# Autodesk Inventor assembly: 14inLift
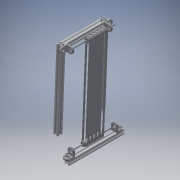
[picture p0: Inventor's stored thumbnail of the model, 180x180]
Saved by Autodesk Inventor 2016 (Build 200138000, 138)
## iProperties
Created: 2016-12-21
Part Number: 14inLift
Document SubType Name: Assembly
Designer: RoboticsUser
Author: RoboticsUser
## Documents named in this file (6)
- C:\Robotics\CAD\2016-17_CAD\14inLift - Copy.iam
- C:\Robotics\CAD\COTSParts\Bosch Extrusion\Bosch 20x20 16.66 -.ipt
- C:\Robotics\CAD\COTSParts\Actobotics\545 parts\545400_MIR.ipt
- C:\Robotics\CAD\COTSParts\Bosch Extrusion\Bosch 20x20 9 in actual.ipt
- C:\Robotics\CAD\2016-17_CAD\12inlift.iam
- C:\Robotics\CAD\COTSParts\Bosch Extrusion\Bosch 20x20 9 real.ipt
## Components (9 placed, 5 different names)
1. Bosch 20x20 16.66 -:1 — Mate:9, Mate:13, Flush:12, Flush:13, Flush:23, Flush:24, Flush:25
2. Bosch 20x20 16.66 -:2 — Mate:12, Mate:14, Flush:16, Flush:17, Flush:20, Flush:21, Flush:22
3. 545400_MIR:1 — Mate:21, Mate:22, Mate:23, Flush:27
4. 545400_MIR:2 — Mate:9, Flush:18, Flush:23
5. 545400_MIR:3 — Mate:19, Flush:19, Mate:20, Flush:26, Flush:28
6. 545400_MIR:4 — Mate:12, Flush:17, Flush:21, Flush:29, Mate:24
7. Bosch 20x20 9 in actual:1 — Mate:13, Flush:12, Flush:13, Mate:14, Flush:16, Flush:18, Flush:20, Flush:22, Flush:24, Flush:25
8. 12inlift:1 [sub-assembly] — Mate:22, Mate:23, Flush:28, Flush:29, Mate:24
9. Bosch 20x20 9 real:1 — Mate:19, Flush:19, Mate:20, Mate:21, Flush:26, Flush:27
## Relationships (26: Flush 16, Mate 10)
- Mate:9: Bosch 20x20 16.66 -:1 ↔ 545400_MIR:2
- Mate:12: Bosch 20x20 16.66 -:2 ↔ 545400_MIR:4
- Mate:13: Bosch 20x20 16.66 -:1 ↔ Bosch 20x20 9 in actual:1
- Flush:12: Bosch 20x20 16.66 -:1 ↔ Bosch 20x20 9 in actual:1
- Flush:13: Bosch 20x20 16.66 -:1 ↔ Bosch 20x20 9 in actual:1
- Mate:14: Bosch 20x20 16.66 -:2 ↔ Bosch 20x20 9 in actual:1
- Flush:16: Bosch 20x20 16.66 -:2 ↔ Bosch 20x20 9 in actual:1
- Flush:17: Bosch 20x20 16.66 -:2 ↔ 545400_MIR:4
- Flush:18: 545400_MIR:2 ↔ Bosch 20x20 9 in actual:1
- Mate:19: 545400_MIR:3 ↔ Bosch 20x20 9 real:1
- Flush:19: 545400_MIR:3 ↔ Bosch 20x20 9 real:1
- Mate:20 (-12.7 mm): 545400_MIR:3 ↔ Bosch 20x20 9 real:1
- Mate:21: 545400_MIR:1 ↔ Bosch 20x20 9 real:1
- Flush:20: Bosch 20x20 16.66 -:2 ↔ Bosch 20x20 9 in actual:1
- Flush:21: Bosch 20x20 16.66 -:2 ↔ 545400_MIR:4
- Flush:22: Bosch 20x20 16.66 -:2 ↔ Bosch 20x20 9 in actual:1
- Flush:23: Bosch 20x20 16.66 -:1 ↔ 545400_MIR:2
- Flush:24: Bosch 20x20 16.66 -:1 ↔ Bosch 20x20 9 in actual:1
- Flush:25: Bosch 20x20 16.66 -:1 ↔ Bosch 20x20 9 in actual:1
- Mate:22: 545400_MIR:1 ↔ 12inlift:1
- Mate:23: 545400_MIR:1 ↔ 12inlift:1
- Flush:26: 545400_MIR:3 ↔ Bosch 20x20 9 real:1
- Flush:27: 545400_MIR:1 ↔ Bosch 20x20 9 real:1
- Flush:28: 545400_MIR:3 ↔ 12inlift:1
- Flush:29 (-25.4 mm): 545400_MIR:4 ↔ 12inlift:1
- Mate:24 (27.432 mm): 545400_MIR:4 ↔ 12inlift:1
